# Autodesk Inventor assembly: Wine Rack Assembly
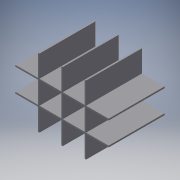
[picture p0: Inventor's stored thumbnail of the model, 180x180]
Saved by Autodesk Inventor 2016 (Build 200138000, 138)
## iProperties
Created: 2017-10-31
Part Number: Wine Rack Assembly
Document SubType Name: Assembly
Designer: mathaetaes
Author: mathaetaes
## Documents named in this file (3)
- E:\Projects\3D Printer\printer projects\My Designs\Bar Cabinet 2.2.2018\Wine Rack Assembly.iam
- E:\Projects\3D Printer\printer projects\My Designs\Bar Cabinet 2.2.2018\Wine Rack Horizontal.ipt
- E:\Projects\3D Printer\printer projects\My Designs\Bar Cabinet 2.2.2018\Wine Rack Vertical.ipt
## Components (5 placed, 2 different names)
1. Wine Rack Horizontal:1 — Flush:1, Mate:1, Mate:3, Mate:8
2. Wine Rack Horizontal:2 — Flush:1, Mate:1, Flush:3, Flush:4, Flush:5, Mate:2, Mate:4, Mate:5, Mate:6, Mate:7
3. Wine Rack Vertical:1 — Flush:3, Mate:6, Mate:7, Mate:8
4. Wine Rack Vertical:2 — Flush:4, Mate:4, Mate:5
5. Wine Rack Vertical:3 — Flush:5, Mate:2, Mate:3
## Relationships (12: Mate 8, Flush 4)
- Flush:1: Wine Rack Horizontal:1 ↔ Wine Rack Horizontal:2
- Mate:1 (88.9 mm): Wine Rack Horizontal:1 ↔ Wine Rack Horizontal:2
- Flush:3: Wine Rack Horizontal:2 ↔ Wine Rack Vertical:1
- Flush:4: Wine Rack Horizontal:2 ↔ Wine Rack Vertical:2
- Flush:5: Wine Rack Horizontal:2 ↔ Wine Rack Vertical:3
- Mate:2: Wine Rack Horizontal:2 ↔ Wine Rack Vertical:3
- Mate:3: Wine Rack Horizontal:1 ↔ Wine Rack Vertical:3
- Mate:4: Wine Rack Horizontal:2 ↔ Wine Rack Vertical:2
- Mate:5: Wine Rack Horizontal:2 ↔ Wine Rack Vertical:2
- Mate:6: Wine Rack Horizontal:2 ↔ Wine Rack Vertical:1
- Mate:7: Wine Rack Horizontal:2 ↔ Wine Rack Vertical:1
- Mate:8: Wine Rack Horizontal:1 ↔ Wine Rack Vertical:1
